# Autodesk Inventor assembly: 1-78.1-79
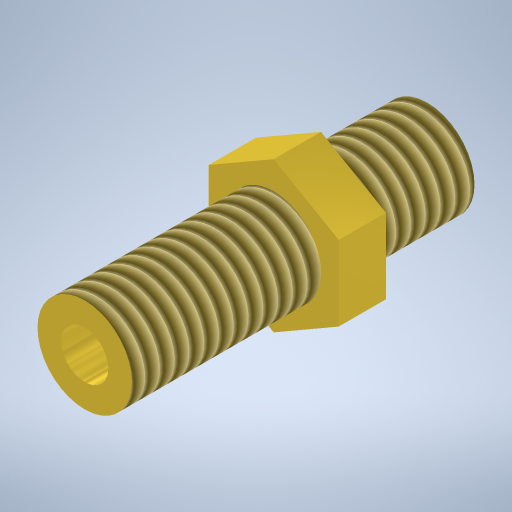
[picture p0: Inventor's stored thumbnail of the model, 512x512]
Saved by Autodesk Inventor 2024.2 (Build 282272000, 272)
## iProperties
Created: 2024-09-29
Part Number: 1-78.1-79
Document SubType Name: Assembly
Designer: melim
Author: melim
## Documents named in this file (3)
- C:\Users\melim\OneDrive\Desktop\PIEZAS_MELISSA\1-78.1-79.iam
- C:\Users\melim\OneDrive\Desktop\PIEZAS_MELISSA\HUDSON-1-78.ipt
- C:\Users\melim\OneDrive\Desktop\PIEZAS_MELISSA\HUDSON-1-79.ipt
## Components (2 placed, 2 different names)
1. HUDSON-1-78:1 — Mate:1, Mate:2
2. HUDSON-1-79:1 — Mate:1, Mate:2
## Relationships (2: Mate 2)
- Mate:1: HUDSON-1-78:1 ↔ HUDSON-1-79:1
- Mate:2 (-16 mm): HUDSON-1-78:1 ↔ HUDSON-1-79:1
